# Autodesk Inventor assembly: Attacker_v1
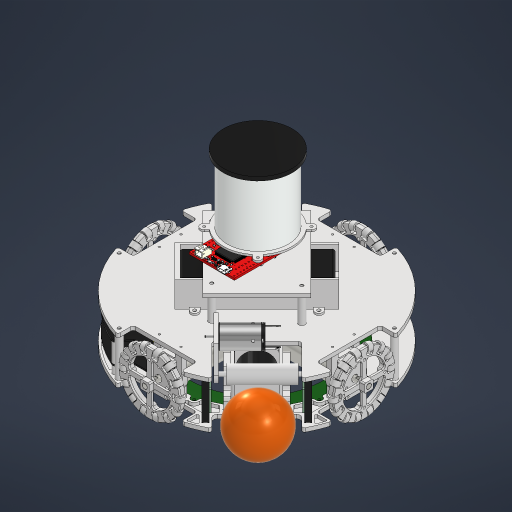
[picture p0: Inventor's stored thumbnail of the model, 512x512]
Saved by Autodesk Inventor 2024.2 (Build 282272000, 272)
## iProperties
Created: 2023-12-21
Part Number: Attacker_v1
Document SubType Name: Assembly
Designer: Hanaoka
Author: Hanaoka
## Documents named in this file (19)
- G:\共有ドライブ\reRo\05_個人\hanaoka\inventor\Attacker_v1.iam
- G:\共有ドライブ\reRo\05_個人\hanaoka\inventor\DriveUnit\DriveUnit.iam
- G:\共有ドライブ\reRo\05_個人\hanaoka\inventor\BasePlate.ipt
- G:\共有ドライブ\reRo\05_個人\hanaoka\inventor\Spacer\Spacer_M2.6x35.ipt
- G:\共有ドライブ\reRo\05_個人\hanaoka\inventor\Ball.ipt
- G:\共有ドライブ\reRo\05_個人\hanaoka\inventor\PCBs\LineSensor_PCB.ipt
- G:\共有ドライブ\reRo\05_個人\hanaoka\inventor\Spacer\Spacer_M2x8.ipt
- G:\共有ドライブ\reRo\05_個人\hanaoka\inventor\PCBs\MainMCU_PCB.ipt
- G:\共有ドライブ\reRo\05_個人\hanaoka\inventor\Spacer\Spacer_M2x15.ipt
- G:\共有ドライブ\reRo\05_個人\hanaoka\inventor\PCBs\MotorDriver_PCB.ipt
- G:\共有ドライブ\reRo\05_個人\hanaoka\inventor\KickerUnit\KickerUnit.iam
- G:\共有ドライブ\reRo\05_個人\hanaoka\inventor\SecondPlate.ipt
- G:\共有ドライブ\reRo\05_個人\hanaoka\inventor\CameraUnit\CameraUnit.iam
- G:\共有ドライブ\reRo\05_個人\hanaoka\inventor\BatteryUnit\BatteryUnit.iam
- G:\共有ドライブ\reRo\05_個人\hanaoka\inventor\DribblerUnit\DribblerUnit.iam
- G:\共有ドライブ\reRo\05_個人\hanaoka\inventor\Spacer\Spacer_M2.6x25.ipt
- G:\共有ドライブ\reRo\05_個人\hanaoka\inventor\ThirdPlate.ipt
- G:\共有ドライブ\reRo\05_個人\hanaoka\inventor\HandleUnit\HandleUnit.iam
- G:\共有ドライブ\reRo\05_個人\hanaoka\inventor\BallSensorUnit\BallSensorUnit.iam
## Components (38 placed, 18 different names)
1. BasePlate:1 — メイト:1, メイト:2, メイト:3, メイト:4, 挿入:1, メイト:5, メイト:6, メイト:7, メイト:8, メイト:9, メイト:10, メイト:11, メイト:12, メイト:13, メイト:14, メイト:15, メイト:16, 挿入:2, 挿入:3, 挿入:4, フラッシュ:1, フラッシュ:2, 挿入:5, 挿入:6, 挿入:7, 挿入:8, メイト:25, メイト:26, メイト:27, メイト:28, メイト:29, メイト:30, メイト:42, メイト:43, メイト:44, メイト:45, メイト:46, メイト:47, メイト:48, メイト:49, メイト:50, メイト:51, メイト:52, メイト:53
2. DriveUnit:1 [sub-assembly] — メイト:2, メイト:3, メイト:4
3. DriveUnit:2 [sub-assembly] — メイト:7, メイト:10, メイト:11
4. DriveUnit:3 [sub-assembly] — メイト:6, メイト:8, メイト:9
5. DriveUnit:4 [sub-assembly] — メイト:5, メイト:12, メイト:13
6. Spacer_M2.6x35:1 — 挿入:1
7. Spacer_M2.6x35:2 — メイト:16, 挿入:3, フラッシュ:5
8. Spacer_M2.6x35:3 — メイト:15, 挿入:4
9. Spacer_M2.6x35:4 — メイト:14, 挿入:2
10. Ball:1
11. LineSensor_PCB:1 — フラッシュ:1, フラッシュ:2
12. Spacer_M2x8:1 — 挿入:5, フラッシュ:3
13. Spacer_M2x8:2 — 挿入:6
14. Spacer_M2x8:3 — 挿入:7
15. Spacer_M2x8:4 — 挿入:8
16. MainMCU_PCB:1 — フラッシュ:3
17. Spacer_M2x15:2
18. Spacer_M2x15:3
19. Spacer_M2x15:4 — フラッシュ:4
20. Spacer_M2x15:1
21. MotorDriver_PCB:1 — フラッシュ:4
22. KickerUnit:1 [sub-assembly] — メイト:25, メイト:26, メイト:27
23. KickerUnit:2 [sub-assembly] — メイト:28, メイト:29, メイト:30
24. SecondPlate:1 — フラッシュ:5, メイト:31, メイト:32, メイト:33, メイト:34, メイト:35, メイト:36, メイト:37, メイト:38, メイト:39, メイト:40, メイト:41
25. CameraUnit:1 [sub-assembly]
26. BatteryUnit:1 [sub-assembly] — メイト:31, メイト:32, メイト:33
27. DribblerUnit:1 [sub-assembly]
28. Spacer_M2.6x25:1 — メイト:34, メイト:38, フラッシュ:6
29. Spacer_M2.6x25:2 — メイト:37, メイト:41
30. Spacer_M2.6x25:3 — メイト:35, メイト:39
31. Spacer_M2.6x25:4 — メイト:36, メイト:40
32. ThirdPlate:1 — フラッシュ:6
33. CameraUnit:2 [sub-assembly]
34. HandleUnit:1 [sub-assembly]
35. BallSensorUnit:1 [sub-assembly] — メイト:43, メイト:51, メイト:53
36. BallSensorUnit:2 [sub-assembly] — メイト:45, メイト:46, メイト:47
37. BallSensorUnit:3 [sub-assembly] — メイト:44, メイト:48, メイト:49
38. BallSensorUnit:4 [sub-assembly] — メイト:42, メイト:50, メイト:52
## Relationships (67: Mate 53, Insert 8, Flush 6)
- メイト:1 [Mate]: BasePlate:1
- メイト:2 [Mate]: BasePlate:1 ↔ DriveUnit:1
- メイト:3 [Mate]: BasePlate:1 ↔ DriveUnit:1
- メイト:4 [Mate]: BasePlate:1 ↔ DriveUnit:1
- 挿入:1 [Insert]: BasePlate:1 ↔ Spacer_M2.6x35:1
- メイト:5 [Mate]: BasePlate:1 ↔ DriveUnit:4
- メイト:6 [Mate]: BasePlate:1 ↔ DriveUnit:3
- メイト:7 [Mate]: BasePlate:1 ↔ DriveUnit:2
- メイト:8 [Mate]: BasePlate:1 ↔ DriveUnit:3
- メイト:9 [Mate]: BasePlate:1 ↔ DriveUnit:3
- メイト:10 [Mate]: BasePlate:1 ↔ DriveUnit:2
- メイト:11 [Mate]: BasePlate:1 ↔ DriveUnit:2
- メイト:12 [Mate]: BasePlate:1 ↔ DriveUnit:4
- メイト:13 [Mate]: BasePlate:1 ↔ DriveUnit:4
- メイト:14 [Mate]: BasePlate:1 ↔ Spacer_M2.6x35:4
- メイト:15 [Mate]: BasePlate:1 ↔ Spacer_M2.6x35:3
- メイト:16 [Mate]: BasePlate:1 ↔ Spacer_M2.6x35:2
- 挿入:2 [Insert]: BasePlate:1 ↔ Spacer_M2.6x35:4
- 挿入:3 [Insert]: BasePlate:1 ↔ Spacer_M2.6x35:2
- 挿入:4 [Insert]: BasePlate:1 ↔ Spacer_M2.6x35:3
- フラッシュ:1 [Flush]: BasePlate:1 ↔ LineSensor_PCB:1
- フラッシュ:2 [Flush]: BasePlate:1 ↔ LineSensor_PCB:1
- 挿入:5 [Insert]: BasePlate:1 ↔ Spacer_M2x8:1
- 挿入:6 [Insert]: BasePlate:1 ↔ Spacer_M2x8:2
- 挿入:7 [Insert]: BasePlate:1 ↔ Spacer_M2x8:3
- 挿入:8 [Insert]: BasePlate:1 ↔ Spacer_M2x8:4
- フラッシュ:3 [Flush]: Spacer_M2x8:1 ↔ MainMCU_PCB:1
- [Mate]: MainMCU_PCB:1 ↔ Spacer_M2x15:3
- [Mate]: MainMCU_PCB:1 ↔ Spacer_M2x15:4
- [Mate]: MainMCU_PCB:1 ↔ Spacer_M2x15:1
- [Mate]: MainMCU_PCB:1 ↔ Spacer_M2x15:2
- [Mate]: MainMCU_PCB:1 ↔ Spacer_M2x15:1
- [Mate]: MainMCU_PCB:1 ↔ Spacer_M2x15:2
- [Mate]: MainMCU_PCB:1 ↔ Spacer_M2x15:3
- [Mate]: MainMCU_PCB:1 ↔ Spacer_M2x15:4
- フラッシュ:4 [Flush]: Spacer_M2x15:4 ↔ MotorDriver_PCB:1
- メイト:25 [Mate]: BasePlate:1 ↔ KickerUnit:1
- メイト:26 [Mate]: BasePlate:1 ↔ KickerUnit:1
- メイト:27 [Mate]: BasePlate:1 ↔ KickerUnit:1
- メイト:28 [Mate]: BasePlate:1 ↔ KickerUnit:2
- メイト:29 [Mate]: BasePlate:1 ↔ KickerUnit:2
- メイト:30 [Mate]: BasePlate:1 ↔ KickerUnit:2
- フラッシュ:5 [Flush]: Spacer_M2.6x35:2 ↔ SecondPlate:1
- メイト:31 [Mate]: SecondPlate:1 ↔ BatteryUnit:1
- メイト:32 [Mate]: SecondPlate:1 ↔ BatteryUnit:1
- メイト:33 [Mate]: SecondPlate:1 ↔ BatteryUnit:1
- メイト:34 [Mate]: SecondPlate:1 ↔ Spacer_M2.6x25:1
- メイト:35 [Mate]: SecondPlate:1 ↔ Spacer_M2.6x25:3
- メイト:36 [Mate]: SecondPlate:1 ↔ Spacer_M2.6x25:4
- メイト:37 [Mate]: SecondPlate:1 ↔ Spacer_M2.6x25:2
- メイト:38 [Mate]: SecondPlate:1 ↔ Spacer_M2.6x25:1
- メイト:39 [Mate]: SecondPlate:1 ↔ Spacer_M2.6x25:3
- メイト:40 [Mate]: SecondPlate:1 ↔ Spacer_M2.6x25:4
- メイト:41 [Mate]: SecondPlate:1 ↔ Spacer_M2.6x25:2
- フラッシュ:6 [Flush]: Spacer_M2.6x25:1 ↔ ThirdPlate:1
- メイト:42 [Mate]: BasePlate:1 ↔ BallSensorUnit:4
- メイト:43 [Mate]: BasePlate:1 ↔ BallSensorUnit:1
- メイト:44 [Mate]: BasePlate:1 ↔ BallSensorUnit:3
- メイト:45 [Mate]: BasePlate:1 ↔ BallSensorUnit:2
- メイト:46 [Mate]: BasePlate:1 ↔ BallSensorUnit:2
- メイト:47 [Mate]: BasePlate:1 ↔ BallSensorUnit:2
- メイト:48 [Mate]: BasePlate:1 ↔ BallSensorUnit:3
- メイト:49 [Mate]: BasePlate:1 ↔ BallSensorUnit:3
- メイト:50 [Mate]: BasePlate:1 ↔ BallSensorUnit:4
- メイト:51 [Mate]: BasePlate:1 ↔ BallSensorUnit:1
- メイト:52 [Mate]: BasePlate:1 ↔ BallSensorUnit:4
- メイト:53 [Mate]: BasePlate:1 ↔ BallSensorUnit:1
